# Autodesk Inventor assembly: 75. Шестерня спидометра ведомая
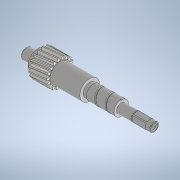
[picture p0: Inventor's stored thumbnail of the model, 180x180]
Saved by Autodesk Inventor 2021 (Build 250183000, 183)
## iProperties
Created: 2021-03-27
Part Number: 75. Шестерня спидометра ведомая
Document SubType Name: Assembly
Designer: Данил
Author: Данил
## Documents named in this file (3)
- C:\Users\Данил\Desktop\Коробка передач\Детали\75. Шестерня спидометра ведомая.iam
- C:\Users\Данил\Desktop\Коробка передач\Детали\75. Шестерня спидометра ведомая.ipt
- C:\Users\Данил\Desktop\Коробка передач\Детали\75. Шестерня спидометра ведомая\Мастер проектирования\Цилиндрическое зубчатое зацепление4.iam
## Components (2 placed, 2 different names)
1. 75. Шестерня спидометра ведомая:1 — Совмещение:1, Заподлицо:1
2. Цилиндрическое зубчатое зацепление:2 [sub-assembly] — Совмещение:1, Заподлицо:1
## Relationships (2: Mate 1, Flush 1)
- Совмещение:1 [Mate]: 75. Шестерня спидометра ведомая:1 ↔ Цилиндрическое зубчатое зацепление:2
- Заподлицо:1 [Flush]: 75. Шестерня спидометра ведомая:1 ↔ Цилиндрическое зубчатое зацепление:2
